# Autodesk Inventor assembly: Conveyor3_FullAssembly
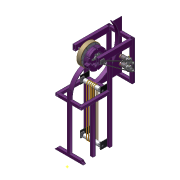
[picture p0: Inventor's stored thumbnail of the model, 180x180]
Saved by Autodesk Inventor 2012 (Build 160160000, 160)
## iProperties
Created: 2012-01-21
Part Number: Conveyor3_FullAssembly
Document SubType Name: Assembly
Designer: JesseK
Mass: 4344.1 g
Surface Area: 18040.8 cm^2
Volume: 2089.73 cm^3
Density: 2.07878 g/cm^3
Author: JesseK
## Documents named in this file (18)
- Z:\UserData\Documents\Inventor\team1885frc\Robot2012\Conveyor3\Conveyor3_FullAssembly.iam
- Z:\UserData\Documents\Inventor\team1885frc\Robot2012\Conveyor3\Frame_Assembly.iam
- Z:\UserData\Documents\Inventor\team1885frc\Robot2012\Conveyor3\Plate_VerticalRollerMount_Top.ipt
- Z:\UserData\Documents\Inventor\team1885frc\Robot2012\Conveyor3\Roller_Top.ipt
- Z:\UserData\Documents\Inventor\team1885frc\Robot2012\Conveyor3\Plate_VerticalRollerMount_Bottom.ipt
- Z:\UserData\Documents\Inventor\team1885frc\Robot2012\Conveyor3\Panel_FrontVerticalConveyorShroud_Lower.ipt
- Z:\UserData\Documents\Inventor\team1885frc\Robot2012\Conveyor3\Belt_VerticalConveyor_Rear.ipt
- Z:\UserData\Documents\Inventor\team1885frc\Robot2012\Conveyor3\Frame_FrontConveyorGuideCurve.ipt
- Z:\UserData\Documents\Inventor\team1885frc\Robot2012\Misc\Generic_Pillow_Block.iam
- Z:\UserData\Documents\Inventor\team1885frc\Hardware\Bolts\Bolt_0.375_16_2.0len_ButtonHead.ipt
- Z:\UserData\Documents\Inventor\team1885frc\Robot2012\Shooter\FlyWheelAssembly3_Jan23.iam
- Z:\UserData\Documents\Inventor\team1885frc\IFI\Imported Components\IFI-WHEEL-ASSY-815-50\IFI-WHEEL-ASSY-815-50.iam
- Z:\UserData\Documents\Inventor\team1885frc\Robot2012\Shooter\ShooterAxle.ipt
- Z:\UserData\Documents\Inventor\team1885frc\Robot2012\Generic_Pillow_Block.ipt
- Z:\UserData\Documents\Inventor\team1885frc\Hardware\Bearings\500id_1.125od_closed_flange_bearing.ipt
- Z:\UserData\Documents\Inventor\team1885frc\Hardware\BeltCogs\Gates_5mmPitch_16T\16 tooth sprocket.iam
- Z:\UserData\Documents\Inventor\team1885frc\Banebots\RS-550_Assembly.iam
- Z:\UserData\Documents\Inventor\team1885frc\Robot2012\Shooter\ShooterBelt.ipt
## Components (36 placed, 16 different names)
1. Frame_Assembly:1 [sub-assembly] — Flush:1, Mate:1, Mate:3, Mate:4, Mate:13, Mate:14, Flush:4, Mate:15, Mate:23, Mate:24, Mate:25, Mate:26, Mate:27, Mate:29, Mate:36, Mate:37, Flush:6, Mate:64, Mate:66, Mate:69, Mate:72, Mate:78, Mate:79, Mate:80
2. Plate_VerticalRollerMount_Top:1 — Flush:1, Mate:1, Mate:3, Flush:2, Flush:3, Mate:45, Mate:48
3. Plate_VerticalRollerMount_Top:2 — Mate:4, Flush:2, Flush:3, Mate:46, Mate:47
4. Roller_Top:1 — Mate:13, Flush:5, Tangent:1, Tangent:2, Tangent:3, Tangent:4, Tangent:5, Tangent:6, Mate:38, Mate:55
5. Roller_Top:2 — Flush:5, Mate:31, Mate:32, Mate:33, Mate:34, Mate:35, Mate:54
6. Plate_VerticalRollerMount_Bottom:1 — Mate:15, Mate:16, Mate:23, Mate:24, Mate:44, Mate:51
7. Plate_VerticalRollerMount_Bottom:2 — Mate:14, Flush:4, Mate:16, Mate:43, Mate:50
8. Panel_FrontVerticalConveyorShroud_Lower:1 — Mate:25, Mate:26, Mate:36
9. Panel_FrontVerticalConveyorShroud_Lower:2 — Mate:27, Mate:29, Mate:37
10. Belt_VerticalConveyor_Rear:1 — Mate:31, Tangent:1, Tangent:5
11. Belt_VerticalConveyor_Rear:2 — Mate:32, Tangent:2
12. Belt_VerticalConveyor_Rear:3 — Mate:33, Tangent:3
13. Belt_VerticalConveyor_Rear:4 — Mate:34, Tangent:4
14. Belt_VerticalConveyor_Rear:5 — Mate:35, Tangent:6
15. Frame_FrontConveyorGuideCurve:1 — Mate:38
16. Generic_Pillow_Block:1 [sub-assembly] — Mate:43, Mate:50, Mate:52, Mate:60, Mate:61
17. Generic_Pillow_Block:2 [sub-assembly] — Mate:44, Mate:51, Mate:52, Mate:53, Mate:54, Mate:62, Mate:63
18. Generic_Pillow_Block:3 [sub-assembly] — Mate:46, Mate:47, Mate:49, Mate:58, Mate:59
19. Generic_Pillow_Block:4 [sub-assembly] — Mate:45, Mate:48, Mate:49, Mate:53, Mate:55, Mate:56, Mate:57
20. Bolt_0.375_16_2.0len_ButtonHead:1 — Mate:58, Mate:59
21. Bolt_0.375_16_2.0len_ButtonHead:2 — Mate:56, Mate:57
22. Bolt_0.375_16_2.0len_ButtonHead:3 — Mate:60, Mate:61
23. Bolt_0.375_16_2.0len_ButtonHead:4 — Mate:62, Mate:63
24. FlyWheelAssembly3_Jan23:1 [sub-assembly] — Mate:65, Mate:66, Mate:68
25. IFI-WHEEL-ASSY-815-50:1 [sub-assembly] — Mate:67, Mate:68
26. ShooterAxle:1 — Flush:6, Mate:64, Mate:65, Mate:67, Mate:70, Mate:71, Mate:77, Flush:7
27. Generic_Pillow_Block:5 — Mate:69, Mate:70, Mate:73, Mate:74
28. Generic_Pillow_Block:6 — Mate:71, Mate:72, Mate:75, Mate:76
29. 500id_1.125od_closed_flange_bearing:1 — Mate:73, Mate:74
30. 500id_1.125od_closed_flange_bearing:2 — Mate:75, Mate:76
31. 16 tooth sprocket:1 [sub-assembly] — Flush:10, Mate:82
32. 16 tooth sprocket:2 [sub-assembly] — Mate:77, Flush:7, Flush:9, Flush:10, Mate:84, Mate:85
33. 16 tooth sprocket:3 [sub-assembly] — Flush:9, Mate:83
34. RS-550_Assembly:1 [sub-assembly] — Mate:78, Flush:8, Mate:80, Mate:81, Mate:82
35. RS-550_Assembly:2 [sub-assembly] — Mate:79, Flush:8, Mate:81, Mate:83
36. ShooterBelt:1 — Mate:84, Mate:85
## Relationships (80: Mate 64, Flush 10, Tangent 6)
- Flush:1: Frame_Assembly:1 ↔ Plate_VerticalRollerMount_Top:1
- Mate:1: Frame_Assembly:1 ↔ Plate_VerticalRollerMount_Top:1
- Mate:3 (3.175 mm): Frame_Assembly:1 ↔ Plate_VerticalRollerMount_Top:1
- Mate:4: Frame_Assembly:1 ↔ Plate_VerticalRollerMount_Top:2
- Flush:2: Plate_VerticalRollerMount_Top:1 ↔ Plate_VerticalRollerMount_Top:2
- Flush:3: Plate_VerticalRollerMount_Top:1 ↔ Plate_VerticalRollerMount_Top:2
- Mate:13 (25.4 mm): Frame_Assembly:1 ↔ Roller_Top:1
- Mate:14: Frame_Assembly:1 ↔ Plate_VerticalRollerMount_Bottom:2
- Flush:4: Frame_Assembly:1 ↔ Plate_VerticalRollerMount_Bottom:2
- Mate:15: Frame_Assembly:1 ↔ Plate_VerticalRollerMount_Bottom:1
- Mate:16: Plate_VerticalRollerMount_Bottom:1 ↔ Plate_VerticalRollerMount_Bottom:2
- Flush:5: Roller_Top:1 ↔ Roller_Top:2
- Mate:23: Frame_Assembly:1 ↔ Plate_VerticalRollerMount_Bottom:1
- Mate:24: Frame_Assembly:1 ↔ Plate_VerticalRollerMount_Bottom:1
- Mate:25: Frame_Assembly:1 ↔ Panel_FrontVerticalConveyorShroud_Lower:1
- Mate:26: Frame_Assembly:1 ↔ Panel_FrontVerticalConveyorShroud_Lower:1
- Mate:27: Frame_Assembly:1 ↔ Panel_FrontVerticalConveyorShroud_Lower:2
- Mate:29: Frame_Assembly:1 ↔ Panel_FrontVerticalConveyorShroud_Lower:2
- Mate:31: Roller_Top:2 ↔ Belt_VerticalConveyor_Rear:1
- Tangent:1: Roller_Top:1 ↔ Belt_VerticalConveyor_Rear:1
- Mate:32: Roller_Top:2 ↔ Belt_VerticalConveyor_Rear:2
- Mate:33: Roller_Top:2 ↔ Belt_VerticalConveyor_Rear:3
- Mate:34: Roller_Top:2 ↔ Belt_VerticalConveyor_Rear:4
- Mate:35: Roller_Top:2 ↔ Belt_VerticalConveyor_Rear:5
- Tangent:2: Roller_Top:1 ↔ Belt_VerticalConveyor_Rear:2
- Tangent:3: Roller_Top:1 ↔ Belt_VerticalConveyor_Rear:3
- Tangent:4: Roller_Top:1 ↔ Belt_VerticalConveyor_Rear:4
- Tangent:5: Roller_Top:1 ↔ Belt_VerticalConveyor_Rear:1
- Tangent:6: Roller_Top:1 ↔ Belt_VerticalConveyor_Rear:5
- Mate:36: Frame_Assembly:1 ↔ Panel_FrontVerticalConveyorShroud_Lower:1
- Mate:37: Frame_Assembly:1 ↔ Panel_FrontVerticalConveyorShroud_Lower:2
- Mate:38: Roller_Top:1 ↔ Frame_FrontConveyorGuideCurve:1
- Mate:43: Plate_VerticalRollerMount_Bottom:2 ↔ Generic_Pillow_Block:1
- Mate:44: Plate_VerticalRollerMount_Bottom:1 ↔ Generic_Pillow_Block:2
- Mate:45: Plate_VerticalRollerMount_Top:1 ↔ Generic_Pillow_Block:4
- Mate:46: Plate_VerticalRollerMount_Top:2 ↔ Generic_Pillow_Block:3
- Mate:47: Plate_VerticalRollerMount_Top:2 ↔ Generic_Pillow_Block:3
- Mate:48: Plate_VerticalRollerMount_Top:1 ↔ Generic_Pillow_Block:4
- Mate:49: Generic_Pillow_Block:3 ↔ Generic_Pillow_Block:4
- Mate:50: Plate_VerticalRollerMount_Bottom:2 ↔ Generic_Pillow_Block:1
- Mate:51: Plate_VerticalRollerMount_Bottom:1 ↔ Generic_Pillow_Block:2
- Mate:52: Generic_Pillow_Block:1 ↔ Generic_Pillow_Block:2
- Mate:53: Generic_Pillow_Block:2 ↔ Generic_Pillow_Block:4
- Mate:54: Roller_Top:2 ↔ Generic_Pillow_Block:2
- Mate:55: Roller_Top:1 ↔ Generic_Pillow_Block:4
- Mate:56: Generic_Pillow_Block:4 ↔ Bolt_0.375_16_2.0len_ButtonHead:2
- Mate:57: Generic_Pillow_Block:4 ↔ Bolt_0.375_16_2.0len_ButtonHead:2
- Mate:58: Generic_Pillow_Block:3 ↔ Bolt_0.375_16_2.0len_ButtonHead:1
- Mate:59: Generic_Pillow_Block:3 ↔ Bolt_0.375_16_2.0len_ButtonHead:1
- Mate:60: Generic_Pillow_Block:1 ↔ Bolt_0.375_16_2.0len_ButtonHead:3
- Mate:61: Generic_Pillow_Block:1 ↔ Bolt_0.375_16_2.0len_ButtonHead:3
- Mate:62: Generic_Pillow_Block:2 ↔ Bolt_0.375_16_2.0len_ButtonHead:4
- Mate:63: Generic_Pillow_Block:2 ↔ Bolt_0.375_16_2.0len_ButtonHead:4
- Flush:6 (-25.4 mm): Frame_Assembly:1 ↔ ShooterAxle:1
- Mate:64: Frame_Assembly:1 ↔ ShooterAxle:1
- Mate:65: FlyWheelAssembly3_Jan23:1 ↔ ShooterAxle:1
- Mate:66 (12.7 mm): Frame_Assembly:1 ↔ FlyWheelAssembly3_Jan23:1
- Mate:67: IFI-WHEEL-ASSY-815-50:1 ↔ ShooterAxle:1
- Mate:68: FlyWheelAssembly3_Jan23:1 ↔ IFI-WHEEL-ASSY-815-50:1
- Mate:69: Frame_Assembly:1 ↔ Generic_Pillow_Block:5
- Mate:70: ShooterAxle:1 ↔ Generic_Pillow_Block:5
- Mate:71: ShooterAxle:1 ↔ Generic_Pillow_Block:6
- Mate:72: Frame_Assembly:1 ↔ Generic_Pillow_Block:6
- Mate:73: Generic_Pillow_Block:5 ↔ 500id_1.125od_closed_flange_bearing:1
- Mate:74: Generic_Pillow_Block:5 ↔ 500id_1.125od_closed_flange_bearing:1
- Mate:75: Generic_Pillow_Block:6 ↔ 500id_1.125od_closed_flange_bearing:2
- Mate:76: Generic_Pillow_Block:6 ↔ 500id_1.125od_closed_flange_bearing:2
- Mate:77: ShooterAxle:1 ↔ 16 tooth sprocket:2
- Flush:7: ShooterAxle:1 ↔ 16 tooth sprocket:2
- Mate:78: Frame_Assembly:1 ↔ RS-550_Assembly:1
- Mate:79: Frame_Assembly:1 ↔ RS-550_Assembly:2
- Flush:8: RS-550_Assembly:1 ↔ RS-550_Assembly:2
- Mate:80: Frame_Assembly:1 ↔ RS-550_Assembly:1
- Mate:81 (25.4 mm): RS-550_Assembly:1 ↔ RS-550_Assembly:2
- Flush:9: 16 tooth sprocket:2 ↔ 16 tooth sprocket:3
- Flush:10: 16 tooth sprocket:1 ↔ 16 tooth sprocket:2
- Mate:82: 16 tooth sprocket:1 ↔ RS-550_Assembly:1
- Mate:83: 16 tooth sprocket:3 ↔ RS-550_Assembly:2
- Mate:84: 16 tooth sprocket:2 ↔ ShooterBelt:1
- Mate:85: 16 tooth sprocket:2 ↔ ShooterBelt:1
